# Autodesk Inventor assembly: I4230
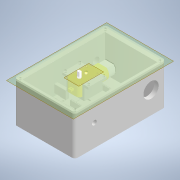
[picture p0: Inventor's stored thumbnail of the model, 180x180]
Saved by Autodesk Inventor 2021 (Build 250183000, 183)
## iProperties
Created: 2020-09-18
Part Number: I4230
Document SubType Name: Assembly
Designer: siwat
Author: siwat
## Documents named in this file (6)
- V:\I4230 OsuTazer\I4230.iam
- V:\I4230 OsuTazer\Motormotor.ipt
- V:\I4230 OsuTazer\TopPlate.ipt
- V:\I4230 OsuTazer\MotorLock.ipt
- V:\I4230 OsuTazer\arduino-yun-1.snapshot.3\Arduino Yun.iam
- V:\I4230 OsuTazer\Base.ipt
## Components (5 placed, 5 different names)
1. Motormotor:1 — Flush:1, Flush:2
2. TopPlate:1 — Flush:1, Flush:2, Flush:3, Flush:4, Flush:5, Flush:6, Flush:7
3. MotorLock:1 — Flush:3, Flush:4, Flush:5
4. Arduino Yun:1 [sub-assembly]
5. Base:1 — Flush:6, Flush:7
## Relationships (7: Flush 7)
- Flush:1: Motormotor:1 ↔ TopPlate:1
- Flush:2: Motormotor:1 ↔ TopPlate:1
- Flush:3: TopPlate:1 ↔ MotorLock:1
- Flush:4: TopPlate:1 ↔ MotorLock:1
- Flush:5: TopPlate:1 ↔ MotorLock:1
- Flush:6: TopPlate:1 ↔ Base:1
- Flush:7: TopPlate:1 ↔ Base:1
